# Autodesk Inventor assembly: Prensa_Hidraulica
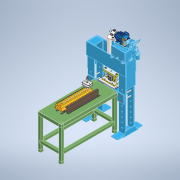
[picture p0: Inventor's stored thumbnail of the model, 180x180]
Saved by Autodesk Inventor 2021 (Build 250183000, 183)
## iProperties
Created: 2020-01-15
Part Number: Prensa_Hidraulica
Document SubType Name: Assembly
Designer: Nelson
Sending System: SolidWorks 2020
Last Author: Micro
Last Saved: 2020-01-16
Author: Nelson
## Documents named in this file (14)
- D:\Nelson\Documentos\Inventor\PrensaHidraulica_Automatizada\Prensa_Hidraulica.iam
- Prensa_Hidraulica.iam
- D:\Nelson\Documentos\Inventor\PrensaHidraulica_Automatizada\Estructura.iam
- D:\Nelson\Documentos\Inventor\PrensaHidraulica_Automatizada\Cilindro neumatico.ipt
- D:\Nelson\Documentos\Inventor\PrensaHidraulica_Automatizada\Bomba Hidraulica.ipt
- D:\Nelson\Documentos\Inventor\PrensaHidraulica_Automatizada\Ensamble Mecanismo cilindro.iam
- D:\Nelson\Documentos\Inventor\PrensaHidraulica_Automatizada\PH 013.ipt
- D:\Nelson\Documentos\Inventor\PrensaHidraulica_Automatizada\Mesa.iam
- D:\Nelson\Documentos\Inventor\PrensaHidraulica_Automatizada\Barra_5-8_950.ipt
- D:\Nelson\Documentos\Inventor\PrensaHidraulica_Automatizada\PerfilZ.ipt
- D:\Nelson\Documentos\Inventor\PrensaHidraulica_Automatizada\Angulo en V.ipt
- D:\Nelson\Documentos\Inventor\PrensaHidraulica_Automatizada\TUBING NOTCHER DIE.iam
- D:\Nelson\Documentos\Inventor\PrensaHidraulica_Automatizada\Soporte de matriz.ipt
- D:\Nelson\Documentos\Inventor\PrensaHidraulica_Automatizada\DIN 7984 - M14 x 35.ipt
## Components (20 placed, 12 different names)
1. Estructura:1 [sub-assembly] — Mate:1, Flush:1, Flush:2, Mate:2, Mate:3, Mate:32, Mate:33, Mate:34, Mate:35, Mate:40, Mate:41, Mate:42, Mate:43, Mate:44, Mate:45, Flush:8, Mate:53, Mate:54, Mate:55
2. Cilindro neumatico:1 — Mate:2, Mate:3
3. Bomba Hidraulica:1 — Mate:1, Flush:1, Flush:2
4. PH 013:3 — Mate:40, Mate:42
5. PH 013:4 — Mate:41, Mate:43
6. PH 013:5 — Mate:34, Mate:35
7. PH 013:6 — Mate:32, Mate:33
8. Ensamble mecanismo cilindro:1 [sub-assembly] — Tangent:1, Tangent:2, Flush:4, Mate:49, Mate:50, Flush:5, Tangent:3, Tangent:4
9. Mesa:1 [sub-assembly] — Mate:44, Mate:45, Flush:4, Mate:47, Mate:48, Flush:6, Flush:7, Flush:8, Mate:63
10. Barra_5-8_950:1 — Tangent:1, Tangent:2, Flush:5
11. PerfilZ:1 — Mate:47, Mate:49
12. PerfilZ:2 — Mate:48, Mate:50
13. Angulo en V:1 — Flush:6, Mate:64
14. Angulo en V:2 — Flush:7, Mate:63, Mate:64, Tangent:3, Tangent:4
15. Soporte de matriz:1 — Mate:53, Mate:54, Mate:55, Mate:56, Mate:57, Mate:58
16. TUBING NOTCHER DIE:1 [sub-assembly] — Mate:56, Mate:57, Mate:58, Mate:59, Flush:9, Mate:60, Flush:10, Mate:61, Flush:11, Mate:62, Flush:12
17. DIN 7984 M14 x 35:1 — Mate:59, Flush:9
18. DIN 7984 M14 x 35:2 — Mate:60, Flush:10
19. DIN 7984 M14 x 35:3 — Mate:62, Flush:12
20. DIN 7984 M14 x 35:4 — Mate:61, Flush:11
## Relationships (44: Mate 29, Flush 11, Tangent 4)
- Mate:1: Estructura:1 ↔ Bomba Hidraulica:1
- Flush:1: Estructura:1 ↔ Bomba Hidraulica:1
- Flush:2: Estructura:1 ↔ Bomba Hidraulica:1
- Mate:2: Estructura:1 ↔ Cilindro neumatico:1
- Mate:3: Estructura:1 ↔ Cilindro neumatico:1
- Mate:32: Estructura:1 ↔ PH 013:6
- Mate:33: Estructura:1 ↔ PH 013:6
- Mate:34: Estructura:1 ↔ PH 013:5
- Mate:35: Estructura:1 ↔ PH 013:5
- Mate:40: Estructura:1 ↔ PH 013:3
- Mate:41: Estructura:1 ↔ PH 013:4
- Mate:42: Estructura:1 ↔ PH 013:3
- Mate:43: Estructura:1 ↔ PH 013:4
- Mate:44: Estructura:1 ↔ Mesa:1
- Mate:45 (25 mm): Estructura:1 ↔ Mesa:1
- Tangent:1: Ensamble mecanismo cilindro:1 ↔ Barra_5-8_950:1
- Tangent:2: Ensamble mecanismo cilindro:1 ↔ Barra_5-8_950:1
- Flush:4 (275 mm): Ensamble mecanismo cilindro:1 ↔ Mesa:1
- Mate:47: Mesa:1 ↔ PerfilZ:1
- Mate:48: Mesa:1 ↔ PerfilZ:2
- Mate:49: Ensamble mecanismo cilindro:1 ↔ PerfilZ:1
- Mate:50: Ensamble mecanismo cilindro:1 ↔ PerfilZ:2
- Flush:5 (-50 mm): Ensamble mecanismo cilindro:1 ↔ Barra_5-8_950:1
- Flush:6: Mesa:1 ↔ Angulo en V:1
- Flush:7: Mesa:1 ↔ Angulo en V:2
- Flush:8: Estructura:1 ↔ Mesa:1
- Mate:53: Estructura:1 ↔ Soporte de matriz:1
- Mate:54: Estructura:1 ↔ Soporte de matriz:1
- Mate:55: Estructura:1 ↔ Soporte de matriz:1
- Mate:56: Soporte de matriz:1 ↔ TUBING NOTCHER DIE:1
- Mate:57: Soporte de matriz:1 ↔ TUBING NOTCHER DIE:1
- Mate:58: Soporte de matriz:1 ↔ TUBING NOTCHER DIE:1
- Mate:59: TUBING NOTCHER DIE:1 ↔ DIN 7984 M14 x 35:1
- Flush:9: TUBING NOTCHER DIE:1 ↔ DIN 7984 M14 x 35:1
- Mate:60: TUBING NOTCHER DIE:1 ↔ DIN 7984 M14 x 35:2
- Flush:10: TUBING NOTCHER DIE:1 ↔ DIN 7984 M14 x 35:2
- Mate:61: TUBING NOTCHER DIE:1 ↔ DIN 7984 M14 x 35:4
- Flush:11: TUBING NOTCHER DIE:1 ↔ DIN 7984 M14 x 35:4
- Mate:62: TUBING NOTCHER DIE:1 ↔ DIN 7984 M14 x 35:3
- Flush:12: TUBING NOTCHER DIE:1 ↔ DIN 7984 M14 x 35:3
- Mate:63 (-296.449 mm): Mesa:1 ↔ Angulo en V:2
- Mate:64 (157.102 mm): Angulo en V:1 ↔ Angulo en V:2
- Tangent:3: Ensamble mecanismo cilindro:1 ↔ Angulo en V:2
- Tangent:4: Ensamble mecanismo cilindro:1 ↔ Angulo en V:2
